# Autodesk Inventor assembly: assyTest
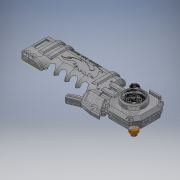
[picture p0: Inventor's stored thumbnail of the model, 180x180]
Saved by Autodesk Inventor 2018 (Build 220112000, 112)
## iProperties
Created: 2019-02-24
Part Number: assyTest
Material: 一般
Document SubType Name: Assembly
Designer: kuwano
Author: kuwano
## Documents named in this file (8)
- D:\Inventor\BayBladeLauncher\parts\assyTest.iam
- D:\Inventor\BayBladeLauncher\parts\bay conect.ipt
- D:\Inventor\BayBladeLauncher\parts\gear.ipt
- D:\Inventor\BayBladeLauncher\parts\undercover1.ipt
- D:\Inventor\BayBladeLauncher\parts\bar.ipt
- D:\Inventor\BayBladeLauncher\parts\joint.ipt
- D:\Inventor\BayBladeLauncher\parts\switch.ipt
- D:\Inventor\BayBladeLauncher\parts\ruber.ipt
## Components (7 placed, 7 different names)
1. bay conect:1 — フラッシュ:1, メイト:5, フラッシュ:2
2. gear:1 — メイト:5, フラッシュ:2
3. undercover1:1 — メイト:1, メイト:2, メイト:3, フラッシュ:1, メイト:6, メイト:12, メイト:19
4. bar:1 — メイト:6, メイト:8, メイト:15, メイト:16, メイト:17, メイト:18, メイト:19
5. joint:1 — メイト:8, メイト:10, メイト:14, メイト:18
6. switch:1 — メイト:10, メイト:12, メイト:14
7. ruber:1 — メイト:15, メイト:16, メイト:17
## Relationships (16: Mate 14, Flush 2)
- メイト:1 [Mate]: undercover1:1
- メイト:2 [Mate]: undercover1:1
- メイト:3 [Mate]: undercover1:1
- フラッシュ:1 [Flush]: bay conect:1 ↔ undercover1:1
- メイト:5 [Mate]: bay conect:1 ↔ gear:1
- フラッシュ:2 [Flush]: bay conect:1 ↔ gear:1
- メイト:6 [Mate]: undercover1:1 ↔ bar:1
- メイト:8 [Mate]: bar:1 ↔ joint:1
- メイト:10 [Mate]: joint:1 ↔ switch:1
- メイト:12 [Mate] (0.5 mm): undercover1:1 ↔ switch:1
- メイト:14 [Mate]: joint:1 ↔ switch:1
- メイト:15 [Mate]: bar:1 ↔ ruber:1
- メイト:16 [Mate]: bar:1 ↔ ruber:1
- メイト:17 [Mate]: bar:1 ↔ ruber:1
- メイト:18 [Mate]: bar:1 ↔ joint:1
- メイト:19 [Mate]: undercover1:1 ↔ bar:1
